# Autodesk Inventor assembly: Bucket - Left (edit)
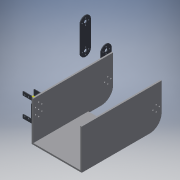
[picture p0: Inventor's stored thumbnail of the model, 180x180]
Saved by Autodesk Inventor 2016 (Build 200138000, 138)
## iProperties
Created: 2015-12-16
Part Number: Bucket - Left (edit)
Document SubType Name: Assembly
Designer: TimB
Author: TimB
## Documents named in this file (4)
- C:\Users\TimB\Documents\GitHub\phi_robotics\3d-models\FTC_Tetrix_KOP_Block_Party\Tim Bloot Designs\JAr JaR Bot\Bucket - Left (edit).iam
- C:\Users\TimB\Documents\GitHub\phi_robotics\3d-models\FTC_Tetrix_KOP_Block_Party\Tetrix_Kit_FTC\Autodesk Inventor Files\tetrix_servo_mount.ipt
- C:\Users\TimB\Documents\GitHub\phi_robotics\3d-models\FTC_Tetrix_KOP_Block_Party\Tim Bloot Designs\JAr JaR Bot\Bucket - Left.ipt
- C:\Users\TimB\Documents\GitHub\phi_robotics\3d-models\FTC_Tetrix_KOP_Block_Party\Tetrix_Kit_FTC\Autodesk Inventor Files\tetrix_739061_2012.ipt
## Components (4 placed, 3 different names)
1. tetrix_servo_mount:1 — Mate:1, Mate:2
2. Bucket - Left:1 — Mate:1, Mate:2, Mate:3, Tangent:1
3. tetrix_739061_2012:1
4. tetrix_739061_2012:2 — Mate:3, Tangent:1
## Relationships (4: Mate 3, Tangent 1)
- Mate:1: tetrix_servo_mount:1 ↔ Bucket - Left:1
- Mate:2: tetrix_servo_mount:1 ↔ Bucket - Left:1
- Mate:3: Bucket - Left:1 ↔ tetrix_739061_2012:2
- Tangent:1: Bucket - Left:1 ↔ tetrix_739061_2012:2
